# Autodesk Inventor assembly: boxx
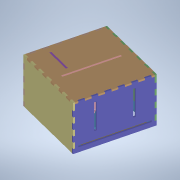
[picture p0: Inventor's stored thumbnail of the model, 180x180]
Saved by Autodesk Inventor 2022 (Build 260153070, 153G)
## iProperties
Created: 2022-05-11
Part Number: boxx
Document SubType Name: Assembly
Designer: Jeanette Guo
Author: Jeanette Guo
## Documents named in this file (9)
- J:\Electronics 3\Message Box\Box\box.iam
- J:\Electronics 3\Message Box\Box\Circuit Cover.ipt
- J:\Electronics 3\Message Box\Box\front.ipt
- J:\Electronics 3\Message Box\Box\sides.ipt
- J:\Electronics 3\Message Box\Box\bottom.ipt
- J:\Electronics 3\Message Box\Box\divider.ipt
- J:\Electronics 3\Message Box\Box\back.ipt
- J:\Electronics 3\Message Box\Box\divider 2.ipt
- J:\Electronics 3\Message Box\Box\shelf.ipt
## Components (9 placed, 8 different names)
1. Circuit Cover:1 — Flush:35
2. sides:1 — Flush:18, Flush:25, Flush:29, Flush:31
3. sides:2 — Flush:19, Flush:23, Flush:24, Flush:26, Flush:28, Flush:30, Mate:4
4. front:1 — Flush:18, Flush:19, Flush:25, Flush:26, Flush:27, Flush:30, Flush:32, Flush:35
5. divider:1 — Mate:4, Flush:33
6. back:1 — Flush:23, Flush:24, Flush:28, Flush:29, Mate:7, Mate:8, Mate:10
7. bottom:1 — Flush:27, Flush:31, Flush:32, Flush:33, Flush:34, Mate:5, Mate:6
8. divider 2:1 — Flush:34, Mate:5, Mate:6, Mate:9
9. shelf:1 — Mate:7, Mate:8, Mate:9, Mate:10
## Relationships (22: Flush 15, Mate 7)
- Flush:18: sides:1 ↔ front:1
- Flush:19: sides:2 ↔ front:1
- Flush:23: sides:2 ↔ back:1
- Flush:24: sides:2 ↔ back:1
- Flush:25: sides:1 ↔ front:1
- Flush:26: sides:2 ↔ front:1
- Flush:27: front:1 ↔ bottom:1
- Flush:28: sides:2 ↔ back:1
- Flush:29: sides:1 ↔ back:1
- Flush:30: sides:2 ↔ front:1
- Flush:31: sides:1 ↔ bottom:1
- Flush:32: front:1 ↔ bottom:1
- Mate:4: sides:2 ↔ divider:1
- Flush:33: divider:1 ↔ bottom:1
- Flush:34: bottom:1 ↔ divider 2:1
- Mate:5: bottom:1 ↔ divider 2:1
- Mate:6: bottom:1 ↔ divider 2:1
- Mate:7: back:1 ↔ shelf:1
- Mate:8: back:1 ↔ shelf:1
- Mate:9: divider 2:1 ↔ shelf:1
- Mate:10: back:1 ↔ shelf:1
- Flush:35: Circuit Cover:1 ↔ front:1
